# Autodesk Inventor assembly: ASY MSC 900.7 support
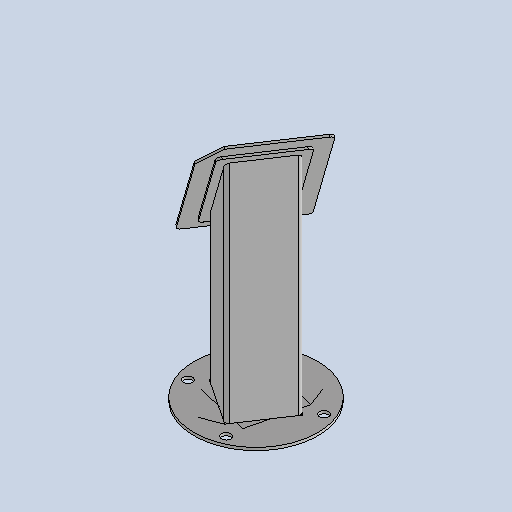
[picture p0: Inventor's stored thumbnail of the model, 512x512]
Saved by Autodesk Inventor 2025.1 (Build 291241020, 241B)
## iProperties
Created: 2024-09-27
Part Number: ASY MSC 900.7 support
Document SubType Name: Assembly
Designer: admin
Author: admin
## Documents named in this file (5)
- C:\Users\user\YandexDisk-badmisterfox\домашниий пк\Inventor\Manturovo\Manturovo_Se-clar\ASY MSC 900.7 support.iam
- C:\Users\user\YandexDisk-badmisterfox\домашниий пк\Inventor\Manturovo\Manturovo_Se-clar\MSC 903 base tube.ipt
- C:\Users\user\YandexDisk-badmisterfox\домашниий пк\Inventor\Manturovo\Manturovo_Se-clar\MSC 904 flange base tube.ipt
- C:\Users\user\YandexDisk-badmisterfox\домашниий пк\Inventor\Manturovo\Manturovo_Se-clar\MSC 905 flange base tube support.ipt
- C:\Users\user\YandexDisk-badmisterfox\домашниий пк\Inventor\Manturovo\Manturovo_Se-clar\MSC 908 tube support 3.ipt
## Components (4 placed, 4 different names)
1. MSC 903 base tube:1 — Rotational:1
2. MSC 904 flange base tube:1 — Rotational:1
3. MSC 905 flange base tube support:1 — Rigid:2
4. MSC 908 tube support 3:1 — Rigid:2
## Relationships (3: WeldJoint 2, RevoluteJoint 1)
- Rotational:1 [RevoluteJoint]: MSC 903 base tube:1 ↔ MSC 904 flange base tube:1
- [WeldJoint]: MSC 903 base tube:1 ↔ MSC 905 flange base tube support:1
- Rigid:2 [WeldJoint]: MSC 905 flange base tube support:1 ↔ MSC 908 tube support 3:1
